# Autodesk Inventor assembly: Flex_SPLINE,REV-ENG
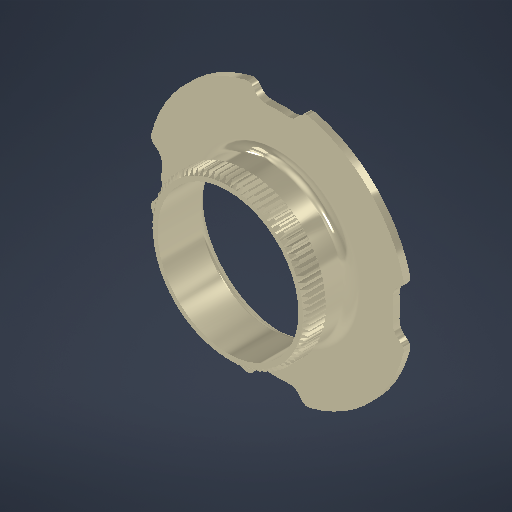
[picture p0: Inventor's stored thumbnail of the model, 512x512]
Saved by Autodesk Inventor 2026.2 (Build 302298010, 298A)
## iProperties
Created: 2026-03-05
Part Number: Flex_SPLINE,REV-ENG
Document SubType Name: Assembly
Designer: 4aida
Author: 4aida
## Documents named in this file (2)
- C:\Users\4aida\OneDrive\Documents\GitHub\Design_II_Group6\REV_ENG\Flex_SPLINE,REV-ENG.iam
- C:\Users\4aida\OneDrive\Documents\GitHub\Design_II_Group6\REV_ENG\Flex_SPLINE,REV-ENG\Design Accelerator\Spur Gears1.iam
## Components (1 placed, 1 different names)
1. Spur Gears:1 [sub-assembly] — Mate:1, Angle:1
## Relationships (2: Mate 1, Angle 1)
- Mate:1: Spur Gears:1
- Angle:1 (0 deg): Spur Gears:1
